# Autodesk Inventor assembly: Pendolo_Inverso
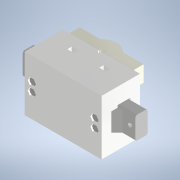
[picture p0: Inventor's stored thumbnail of the model, 180x180]
Saved by Autodesk Inventor 2020.2 (Build 242310000, 310)
## iProperties
Created: 2019-11-10
Part Number: Pendolo_Inverso
Document SubType Name: Assembly
Designer: socci
Author: socci
## Documents named in this file (10)
- C:\Users\socci\Desktop\mv-Project\04_PartDraw\Assieme_Base.iam
- C:\Users\socci\Desktop\mv-Project\04_PartDraw\Componenti\19_Base_Pezzo_Unico.ipt
- C:\Users\socci\Desktop\mv-Project\04_PartDraw\Componenti\20_Base_Sopra.ipt
- C:\Users\socci\Desktop\mv-Project\04_PartDraw\Componenti\22_Blocco_Escursione_Braccio.ipt
- C:\Users\socci\Documents\Inventor\Content Center Files\R2020\it-IT\UNI 5739\UNI 5739 - M5 x 40.ipt
- C:\Users\socci\Documents\Inventor\Content Center Files\R2020\it-IT\IS 2016  A\IS 2016 - A5,5.ipt
- C:\Users\socci\Documents\Inventor\Content Center Files\R2020\it-IT\AS 1112 (4)\AS 1112 - M5(2).ipt
- C:\Users\socci\Documents\Inventor\Content Center Files\R2020\it-IT\UNI 5739\UNI 5739 - M6 x 60.ipt
- C:\Users\socci\Documents\Inventor\Content Center Files\R2020\it-IT\AS 1112 (2)\AS 1112 - M6  Tipo 5.ipt
- C:\Users\socci\Documents\Inventor\Content Center Files\R2020\it-IT\IS 2016  A\IS 2016 - A6,6.ipt
## Components (33 placed, 9 different names)
1. 19_Base_Pezzo_Unico:1 — Coincidente:3, Coincidente:4, Coincidente:11, Coincidente:12, Allineato:4, Coincidente:14, Coincidente:15, Allineato:5, Inserimento:323, Inserimento:327, Inserimento:331, Inserimento:335, Coincidente:28, Inserimento:365, Inserimento:368, Coincidente:33, Coincidente:34, Inserimento:371, Inserimento:372, Inserimento:374, Inserimento:376
2. 20_Base_Sopra:1 — Coincidente:3, Inserimento:321, Inserimento:322, Inserimento:325, Inserimento:326
3. 20_Base_Sopra:2 — Coincidente:4, Inserimento:329, Inserimento:330, Inserimento:333, Inserimento:334
4. 22_Blocco_Escursione_Braccio:1 — Coincidente:11, Coincidente:12, Allineato:4
5. 22_Blocco_Escursione_Braccio:2 — Coincidente:14, Coincidente:15, Allineato:5
6. UNI 5739 M6 x 60:5
7. IS 2016 A A6,6:5 — Inserimento:374
8. UNI 5739 M6 x 60:6
9. IS 2016 A A6,6:6 — Inserimento:376
10. UNI 5739 M6 x 60:3
11. AS 1112 (2) - Metrico M6  Tipo 5:3 — Coincidente:34
12. IS 2016 A A6,6:3 — Coincidente:33
13. UNI 5739 M6 x 60:4
14. AS 1112 (2) - Metrico M6  Tipo 5:4 — Inserimento:372
15. IS 2016 A A6,6:4 — Inserimento:371
16. AS 1112 (2) - Metrico M6  Tipo 5:2 — Inserimento:368
17. AS 1112 (2) - Metrico M6  Tipo 5:1 — Inserimento:365
18. UNI 5739 M5 x 40:4 — Inserimento:320
19. IS 2016 A A5,5:7 — Inserimento:322
20. IS 2016 A A5,5:8 — Inserimento:320, Inserimento:321
21. AS 1112 (4) - Metrico M5:1 — Inserimento:323
22. UNI 5739 M5 x 40:5
23. IS 2016 A A5,5:9 — Inserimento:326
24. IS 2016 A A5,5:10 — Inserimento:325
25. AS 1112 (4) - Metrico M5:2 — Inserimento:327
26. UNI 5739 M5 x 40:6
27. IS 2016 A A5,5:11 — Inserimento:330
28. IS 2016 A A5,5:12 — Inserimento:329
29. AS 1112 (4) - Metrico M5:3 — Inserimento:331
30. UNI 5739 M5 x 40:7
31. IS 2016 A A5,5:13 — Inserimento:334
32. IS 2016 A A5,5:14 — Inserimento:333
33. AS 1112 (4) - Metrico M5:4 — Inserimento:335
## Relationships (37: Insert 26, Mate 9, Flush 2)
- Coincidente:3 [Mate] (1 mm): 19_Base_Pezzo_Unico:1 ↔ 20_Base_Sopra:1
- Coincidente:4 [Mate] (1 mm): 19_Base_Pezzo_Unico:1 ↔ 20_Base_Sopra:2
- Coincidente:11 [Mate]: 19_Base_Pezzo_Unico:1 ↔ 22_Blocco_Escursione_Braccio:1
- Coincidente:12 [Mate] (0.2 mm): 19_Base_Pezzo_Unico:1 ↔ 22_Blocco_Escursione_Braccio:1
- Allineato:4 [Flush]: 19_Base_Pezzo_Unico:1 ↔ 22_Blocco_Escursione_Braccio:1
- Coincidente:14 [Mate] (0.2 mm): 19_Base_Pezzo_Unico:1 ↔ 22_Blocco_Escursione_Braccio:2
- Coincidente:15 [Mate]: 19_Base_Pezzo_Unico:1 ↔ 22_Blocco_Escursione_Braccio:2
- Allineato:5 [Flush]: 19_Base_Pezzo_Unico:1 ↔ 22_Blocco_Escursione_Braccio:2
- Inserimento:320: UNI 5739 M5 x 40:4 ↔ IS 2016 A A5,5:8
- Inserimento:321: 20_Base_Sopra:1 ↔ IS 2016 A A5,5:8
- Inserimento:322: 20_Base_Sopra:1 ↔ IS 2016 A A5,5:7
- Inserimento:323: 19_Base_Pezzo_Unico:1 ↔ AS 1112 (4) - Metrico M5:1
- [Insert]: UNI 5739 M5 x 40:5 ↔ IS 2016 A A5,5:10
- Inserimento:325: 20_Base_Sopra:1 ↔ IS 2016 A A5,5:10
- Inserimento:326: 20_Base_Sopra:1 ↔ IS 2016 A A5,5:9
- Inserimento:327: 19_Base_Pezzo_Unico:1 ↔ AS 1112 (4) - Metrico M5:2
- [Insert]: UNI 5739 M5 x 40:6 ↔ IS 2016 A A5,5:12
- Inserimento:329: 20_Base_Sopra:2 ↔ IS 2016 A A5,5:12
- Inserimento:330: 20_Base_Sopra:2 ↔ IS 2016 A A5,5:11
- Inserimento:331: 19_Base_Pezzo_Unico:1 ↔ AS 1112 (4) - Metrico M5:3
- [Insert]: UNI 5739 M5 x 40:7 ↔ IS 2016 A A5,5:14
- Inserimento:333: 20_Base_Sopra:2 ↔ IS 2016 A A5,5:14
- Inserimento:334: 20_Base_Sopra:2 ↔ IS 2016 A A5,5:13
- Inserimento:335: 19_Base_Pezzo_Unico:1 ↔ AS 1112 (4) - Metrico M5:4
- Coincidente:28 [Mate]: 19_Base_Pezzo_Unico:1
- Inserimento:365: 19_Base_Pezzo_Unico:1 ↔ AS 1112 (2) - Metrico M6  Tipo 5:1
- Inserimento:368: 19_Base_Pezzo_Unico:1 ↔ AS 1112 (2) - Metrico M6  Tipo 5:2
- [Insert]: UNI 5739 M6 x 60:3 ↔ IS 2016 A A6,6:3
- Coincidente:33 [Mate]: 19_Base_Pezzo_Unico:1 ↔ IS 2016 A A6,6:3
- Coincidente:34 [Mate]: 19_Base_Pezzo_Unico:1 ↔ AS 1112 (2) - Metrico M6  Tipo 5:3
- [Insert]: UNI 5739 M6 x 60:4 ↔ IS 2016 A A6,6:4
- Inserimento:371: 19_Base_Pezzo_Unico:1 ↔ IS 2016 A A6,6:4
- Inserimento:372: 19_Base_Pezzo_Unico:1 ↔ AS 1112 (2) - Metrico M6  Tipo 5:4
- [Insert]: UNI 5739 M6 x 60:5 ↔ IS 2016 A A6,6:5
- Inserimento:374: 19_Base_Pezzo_Unico:1 ↔ IS 2016 A A6,6:5
- [Insert]: UNI 5739 M6 x 60:6 ↔ IS 2016 A A6,6:6
- Inserimento:376: 19_Base_Pezzo_Unico:1 ↔ IS 2016 A A6,6:6
## Named parameters: d522_d518 = 0 mm, d526_d518 = 0 mm, d530_d518 = 0 mm, d592_d586 = 0 mm, d595_d586 = 0 mm, d604_d592_d586 = 0 mm, d606_d592_d586 = 0 mm
